# Autodesk Inventor assembly: Table
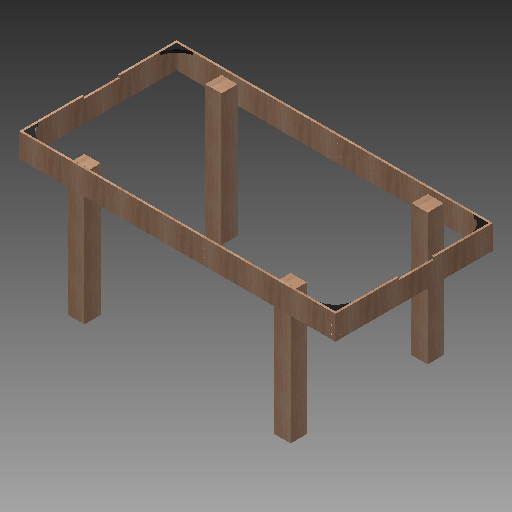
[picture p0: Inventor's stored thumbnail of the model, 512x512]
Saved by Autodesk Inventor 2019.3 (Build 233278000, 278)
## iProperties
Created: 2020-08-13
Part Number: Table
Material: Generisch
Document SubType Name: Assembly
Designer: Nicolas Frick
Author: Nicolas Frick
## Documents named in this file (4)
- C:\Users\Nicolas Frick\Sync\OneDrive\airhockeybot\mechanical_design\inventor\Table\Table.iam
- C:\Users\Nicolas Frick\Sync\OneDrive\airhockeybot\mechanical_design\inventor\Table\Frame.ipt
- C:\Users\Nicolas Frick\Sync\OneDrive\airhockeybot\mechanical_design\inventor\Table\Leg.ipt
- C:\Users\Nicolas Frick\Sync\OneDrive\airhockeybot\mechanical_design\inventor\Corner.ipt
## Components (9 placed, 3 different names)
1. Frame:1 — Passend:7, Passend:8, Passend:9, Passend:10, Passend:11, Passend:12, Passend:13, Passend:14, Passend:18, Passend:19, Passend:20, Passend:21, Passend:22, Passend:23, Passend:24, Passend:25
2. Leg:1 — Passend:7, Passend:12
3. Leg:2 — Passend:8, Passend:11
4. Leg:3 — Passend:10, Passend:14
5. Leg:4 — Passend:9, Passend:13
6. Corner:1 — Passend:24, Passend:25
7. Corner:2 — Passend:20, Passend:23
8. Corner:3 — Passend:19, Passend:21
9. Corner:4 — Passend:18, Passend:22
## Relationships (16: Mate 16)
- Passend:7 [Mate]: Frame:1 ↔ Leg:1
- Passend:8 [Mate]: Frame:1 ↔ Leg:2
- Passend:9 [Mate]: Frame:1 ↔ Leg:4
- Passend:10 [Mate]: Frame:1 ↔ Leg:3
- Passend:11 [Mate] (259 mm): Frame:1 ↔ Leg:2
- Passend:12 [Mate] (259 mm): Frame:1 ↔ Leg:1
- Passend:13 [Mate] (259 mm): Frame:1 ↔ Leg:4
- Passend:14 [Mate] (259 mm): Frame:1 ↔ Leg:3
- Passend:18 [Mate]: Frame:1 ↔ Corner:4
- Passend:19 [Mate]: Frame:1 ↔ Corner:3
- Passend:20 [Mate]: Frame:1 ↔ Corner:2
- Passend:21 [Mate]: Frame:1 ↔ Corner:3
- Passend:22 [Mate]: Frame:1 ↔ Corner:4
- Passend:23 [Mate]: Frame:1 ↔ Corner:2
- Passend:24 [Mate]: Frame:1 ↔ Corner:1
- Passend:25 [Mate]: Frame:1 ↔ Corner:1
